# Autodesk Inventor assembly: ADXL_345_CaseAssembly
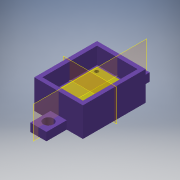
[picture p0: Inventor's stored thumbnail of the model, 180x180]
Saved by Autodesk Inventor 2016 SP1 (Build 200210100, 210)
## iProperties
Created: 2016-02-02
Part Number: ADXL_345_CaseAssembly
Document SubType Name: Assembly
Designer: steele
Author: steele
## Documents named in this file (3)
- C:\snobotics\CAD-Development\robSteele\SnoBotics2016\AM Parts\ADXL_345_CaseAssembly.iam
- C:\snobotics\CAD-Development\robSteele\SnoBotics2016\AM Parts\CaseForADXL_345.ipt
- C:\snobotics\CAD-Development\robSteele\SnoBotics2016\AM Parts\ADXL_345.ipt
## Components (2 placed, 2 different names)
1. CaseForADXL_345:1 — Mate:1, Mate:2, Mate:3
2. ADXL_345:1 — Mate:1, Mate:2, Mate:3
## Relationships (3: Mate 3)
- Mate:1: CaseForADXL_345:1 ↔ ADXL_345:1
- Mate:2: CaseForADXL_345:1 ↔ ADXL_345:1
- Mate:3: CaseForADXL_345:1 ↔ ADXL_345:1
